# Autodesk Inventor assembly: MG_996R
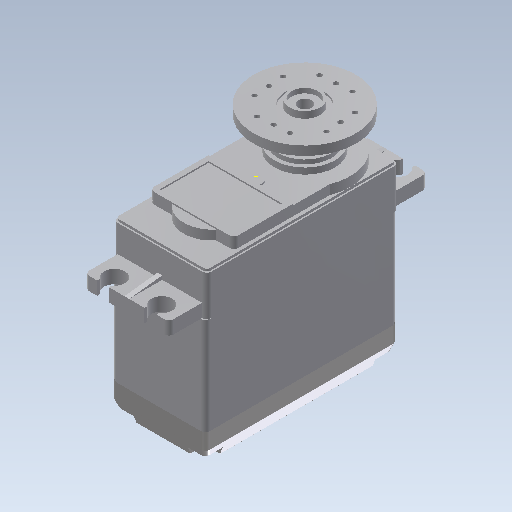
[picture p0: Inventor's stored thumbnail of the model, 512x512]
Saved by Autodesk Inventor 2020 (Build 240168000, 168)
## iProperties
Created: 2016-09-26
Part Number: MG_996R
Document SubType Name: Assembly
Designer: Julian
Author: Julian
## Documents named in this file (6)
- C:\Users\Gebruiker\Documents\GitHub\BeerMinder\3D-model\servo\MG_996R.iam
- C:\Users\Gebruiker\Documents\GitHub\BeerMinder\3D-model\servo\Base.ipt
- C:\Users\Gebruiker\Documents\GitHub\BeerMinder\3D-model\servo\Medio.ipt
- C:\Users\Gebruiker\Documents\GitHub\BeerMinder\3D-model\servo\Top.ipt
- C:\Users\Gebruiker\Documents\GitHub\BeerMinder\3D-model\servo\Eje.ipt
- C:\Users\Gebruiker\Documents\GitHub\BeerMinder\3D-model\servo\Acople circular.ipt
## Components (5 placed, 5 different names)
1. Top:1 — Rígido:2, De rotación:1
2. Medio:1 — Rígido:1, Rígido:2
3. Base:1 — Rígido:1
4. Eje:1 — De rotación:1, De rotación:2
5. Acople circular:1 — De rotación:2
## Relationships (4: WeldJoint 2, RevoluteJoint 2)
- Rígido:1 [WeldJoint]: Medio:1 ↔ Base:1
- Rígido:2 [WeldJoint]: Top:1 ↔ Medio:1
- De rotación:1 [RevoluteJoint]: Top:1 ↔ Eje:1
- De rotación:2 [RevoluteJoint]: Eje:1 ↔ Acople circular:1
